# Autodesk Inventor assembly: base
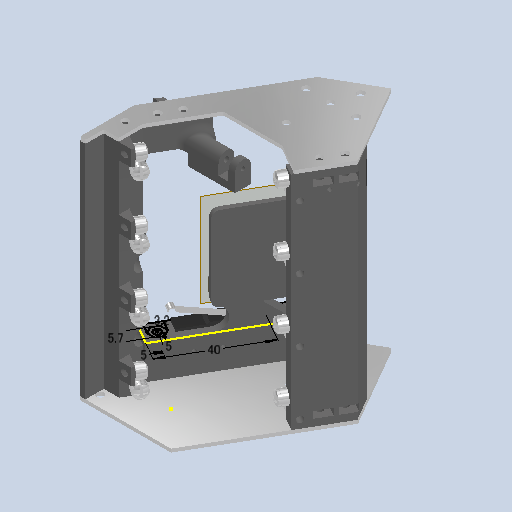
[picture p0: Inventor's stored thumbnail of the model, 512x512]
Saved by Autodesk Inventor 2024.1 (Build 281209000, 209)
## iProperties
Created: 2025-01-17
Part Number: base
Document SubType Name: Assembly
Designer: hibik
Author: hibik
## Documents named in this file (8)
- C:\Users\hibik\Documents\Robomech\RESCUE\ORCA\hard\fork\right\base.iam
- C:\Users\hibik\Documents\Robomech\RESCUE\ORCA\hard\fork\right\base_base.ipt
- C:\Users\hibik\Documents\Robomech\RESCUE\ORCA\hard\std_parts\bearing_3_6_2.5.ipt
- C:\Users\hibik\Documents\Robomech\RESCUE\ORCA\hard\fork\right\base_bearingpole_side.ipt
- C:\Users\hibik\Documents\Robomech\RESCUE\ORCA\hard\fork\right\base_cover.ipt
- C:\Users\hibik\Documents\Robomech\RESCUE\ORCA\hard\fork\right\limit_setter_under.ipt
- C:\Users\hibik\Documents\Robomech\RESCUE\ORCA\hard\std_parts\limit_switch.ipt
- C:\Users\hibik\Documents\Robomech\RESCUE\ORCA\hard\fork\right\base_bearingpole_front_assy.iam
## Components (23 placed, 7 different names)
1. base_base:1 — メイト:2, フラッシュ:3, フラッシュ:4, フラッシュ:5, フラッシュ:6, フラッシュ:7, メイト:4, 挿入:21
2. bearing_3_6_2.5:1 — 挿入:31
3. bearing_3_6_2.5:2 — 挿入:30
4. bearing_3_6_2.5:3 — 挿入:29
5. bearing_3_6_2.5:4 — 挿入:28
6. bearing_3_6_2.5:5 — 挿入:27
7. bearing_3_6_2.5:6 — 挿入:26
8. bearing_3_6_2.5:7 — 挿入:24
9. bearing_3_6_2.5:8 — 挿入:25
10. base_bearingpole_side:1 — メイト:2, フラッシュ:3, フラッシュ:4, 挿入:9, 挿入:10, 挿入:11, 挿入:12, 挿入:13, 挿入:14, 挿入:15, 挿入:16, メイト:3, 挿入:19, 挿入:20
11. bearing_3_6_2.5:9 — 挿入:9
12. bearing_3_6_2.5:10 — 挿入:10
13. bearing_3_6_2.5:11 — 挿入:11
14. bearing_3_6_2.5:12 — 挿入:12
15. bearing_3_6_2.5:13 — 挿入:13
16. bearing_3_6_2.5:14 — 挿入:14
17. bearing_3_6_2.5:15 — 挿入:15
18. bearing_3_6_2.5:16 — 挿入:16
19. base_cover:1 — メイト:3, フラッシュ:5, フラッシュ:6, 挿入:22, 挿入:23
20. limit_setter_under:1 — フラッシュ:7, メイト:4, 挿入:17, 挿入:18
21. limit_switch:1 — 挿入:17, 挿入:18
22. limit_switch:2 — 挿入:19, 挿入:20
23. base_bearingpole_front_assy:1 [sub-assembly] — 挿入:21, 挿入:22, 挿入:23, 挿入:24, 挿入:25, 挿入:26, 挿入:27, 挿入:28, 挿入:29, 挿入:30, 挿入:31
## Relationships (31: Insert 23, Flush 5, Mate 3)
- メイト:2 [Mate]: base_base:1 ↔ base_bearingpole_side:1
- フラッシュ:3 [Flush]: base_base:1 ↔ base_bearingpole_side:1
- フラッシュ:4 [Flush]: base_base:1 ↔ base_bearingpole_side:1
- 挿入:9 [Insert]: base_bearingpole_side:1 ↔ bearing_3_6_2.5:9
- 挿入:10 [Insert]: base_bearingpole_side:1 ↔ bearing_3_6_2.5:10
- 挿入:11 [Insert]: base_bearingpole_side:1 ↔ bearing_3_6_2.5:11
- 挿入:12 [Insert]: base_bearingpole_side:1 ↔ bearing_3_6_2.5:12
- 挿入:13 [Insert]: base_bearingpole_side:1 ↔ bearing_3_6_2.5:13
- 挿入:14 [Insert]: base_bearingpole_side:1 ↔ bearing_3_6_2.5:14
- 挿入:15 [Insert]: base_bearingpole_side:1 ↔ bearing_3_6_2.5:15
- 挿入:16 [Insert]: base_bearingpole_side:1 ↔ bearing_3_6_2.5:16
- メイト:3 [Mate]: base_bearingpole_side:1 ↔ base_cover:1
- フラッシュ:5 [Flush]: base_base:1 ↔ base_cover:1
- フラッシュ:6 [Flush]: base_base:1 ↔ base_cover:1
- フラッシュ:7 [Flush]: base_base:1 ↔ limit_setter_under:1
- メイト:4 [Mate]: base_base:1 ↔ limit_setter_under:1
- 挿入:17 [Insert]: limit_setter_under:1 ↔ limit_switch:1
- 挿入:18 [Insert]: limit_setter_under:1 ↔ limit_switch:1
- 挿入:19 [Insert]: base_bearingpole_side:1 ↔ limit_switch:2
- 挿入:20 [Insert]: base_bearingpole_side:1 ↔ limit_switch:2
- 挿入:21 [Insert]: base_base:1 ↔ base_bearingpole_front_assy:1
- 挿入:22 [Insert]: base_cover:1 ↔ base_bearingpole_front_assy:1
- 挿入:23 [Insert]: base_cover:1 ↔ base_bearingpole_front_assy:1
- 挿入:24 [Insert]: bearing_3_6_2.5:7 ↔ base_bearingpole_front_assy:1
- 挿入:25 [Insert]: bearing_3_6_2.5:8 ↔ base_bearingpole_front_assy:1
- 挿入:26 [Insert]: bearing_3_6_2.5:6 ↔ base_bearingpole_front_assy:1
- 挿入:27 [Insert]: bearing_3_6_2.5:5 ↔ base_bearingpole_front_assy:1
- 挿入:28 [Insert]: bearing_3_6_2.5:4 ↔ base_bearingpole_front_assy:1
- 挿入:29 [Insert]: bearing_3_6_2.5:3 ↔ base_bearingpole_front_assy:1
- 挿入:30 [Insert]: bearing_3_6_2.5:2 ↔ base_bearingpole_front_assy:1
- 挿入:31 [Insert]: bearing_3_6_2.5:1 ↔ base_bearingpole_front_assy:1
